# Autodesk Inventor assembly: Hopper Assembly
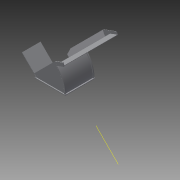
[picture p0: Inventor's stored thumbnail of the model, 180x180]
Saved by Autodesk Inventor 2013 (Build 170138000, 138)
## iProperties
Created: 2013-01-27
Part Number: Hopper Assembly
Document SubType Name: Assembly
Designer: Andrew Toennies
Mass: 1217.41 g
Surface Area: 7062.66 cm^2
Volume: 1014.51 cm^3
Density: 1.2 g/cm^3
Author: Andrew Toennies
## Documents named in this file (13)
- C:\Users\Moses\Documents\GitHub\frc2013CAD\Launcher\Hopper New\Hopper Assembly.iam
- C:\Users\Moses\Documents\GitHub\frc2013CAD\Launcher\Hopper New\Bottom Plate.ipt
- C:\Users\Moses\Documents\GitHub\frc2013CAD\Launcher\Hopper New\Outer Rail.ipt
- C:\Users\Moses\Documents\GitHub\frc2013CAD\Launcher\Hopper New\Inner Rail.ipt
- C:\Users\Moses\Documents\GitHub\frc2013CAD\Launcher\Hopper New\Side Panel.ipt
- C:\Users\Moses\Documents\GitHub\frc2013CAD\Launcher\Hopper New\Side Panel 2.ipt
- C:\Users\Moses\Documents\GitHub\frc2013CAD\Launcher\Hopper New\Wing.ipt
- C:\Users\Moses\Documents\GitHub\frc2013CAD\Launcher\Hopper New\Top.ipt
- C:\Users\Moses\Documents\GitHub\frc2013CAD\Launcher\Hopper New\Backboard.ipt
- C:\Users\Moses\Documents\GitHub\frc2013CAD\Launcher\Hopper New\Mount.ipt
- C:\Users\Moses\Documents\GitHub\frc2013CAD\Launcher\Hopper New\Side Wall.ipt
- C:\Users\Moses\Documents\GitHub\frc2013CAD\Launcher\Hopper New\Side Wall 2.ipt
- C:\Users\Moses\Documents\GitHub\frc2013CAD\Launcher\Hopper New\Back.ipt
## Components (12 placed, 12 different names)
1. Bottom Plate:1 — Flush:5, Mate:20, Mate:22, Mate:25, Mate:26, Mate:29, Mate:36, Mate:39, Flush:8, Mate:40, Mate:41, Mate:42, Flush:11, Mate:51
2. Outer Rail:3 — Flush:5, Mate:20, Mate:22, Mate:28
3. Side Panel:1 — Mate:25, Mate:26, Mate:32, Mate:33, Mate:37, Flush:7
4. Side Panel 2:3 — Mate:28, Mate:29, Mate:36, Mate:49, Mate:50
5. Top:1 — Mate:32, Mate:33, Mate:35, Mate:38, Flush:7, Flush:9, Mate:47, Flush:14, Mate:48
6. Backboard:1 — Mate:37, Mate:38, Flush:10
7. Inner Rail:1 — Mate:39, Flush:8, Mate:40, Flush:9, Flush:10, Flush:12, Mate:43, Mate:44
8. Mount:1 — Mate:41, Mate:42, Flush:11
9. Wing:1 — Flush:12, Mate:43, Mate:44, Mate:45, Flush:13, Mate:46
10. Side Wall:1 — Mate:45, Flush:13, Mate:46
11. Side Wall 2:1 — Mate:47, Flush:14, Mate:48
12. Back:1 — Mate:49, Mate:50, Mate:51
## Relationships (34: Mate 25, Flush 9)
- Flush:5: Bottom Plate:1 ↔ Outer Rail:3
- Mate:20: Bottom Plate:1 ↔ Outer Rail:3
- Mate:22: Bottom Plate:1 ↔ Outer Rail:3
- Mate:25: Bottom Plate:1 ↔ Side Panel:1
- Mate:26: Bottom Plate:1 ↔ Side Panel:1
- Mate:28: Outer Rail:3 ↔ Side Panel 2:3
- Mate:29: Bottom Plate:1 ↔ Side Panel 2:3
- Mate:32: Side Panel:1 ↔ Top:1
- Mate:33 (3.175 mm): Side Panel:1 ↔ Top:1
- Mate:35: Top:1
- Mate:36: Bottom Plate:1 ↔ Side Panel 2:3
- Mate:37: Side Panel:1 ↔ Backboard:1
- Mate:38: Top:1 ↔ Backboard:1
- Flush:7: Side Panel:1 ↔ Top:1
- Mate:39: Bottom Plate:1 ↔ Inner Rail:1
- Flush:8: Bottom Plate:1 ↔ Inner Rail:1
- Mate:40: Bottom Plate:1 ↔ Inner Rail:1
- Flush:9: Top:1 ↔ Inner Rail:1
- Flush:10: Backboard:1 ↔ Inner Rail:1
- Mate:41: Bottom Plate:1 ↔ Mount:1
- Mate:42: Bottom Plate:1 ↔ Mount:1
- Flush:11: Bottom Plate:1 ↔ Mount:1
- Flush:12: Inner Rail:1 ↔ Wing:1
- Mate:43: Inner Rail:1 ↔ Wing:1
- Mate:44: Inner Rail:1 ↔ Wing:1
- Mate:45: Wing:1 ↔ Side Wall:1
- Flush:13: Wing:1 ↔ Side Wall:1
- Mate:46: Wing:1 ↔ Side Wall:1
- Mate:47: Top:1 ↔ Side Wall 2:1
- Flush:14: Top:1 ↔ Side Wall 2:1
- Mate:48: Top:1 ↔ Side Wall 2:1
- Mate:49: Side Panel 2:3 ↔ Back:1
- Mate:50: Side Panel 2:3 ↔ Back:1
- Mate:51: Bottom Plate:1 ↔ Back:1
